# Autodesk Inventor assembly: Assembly1
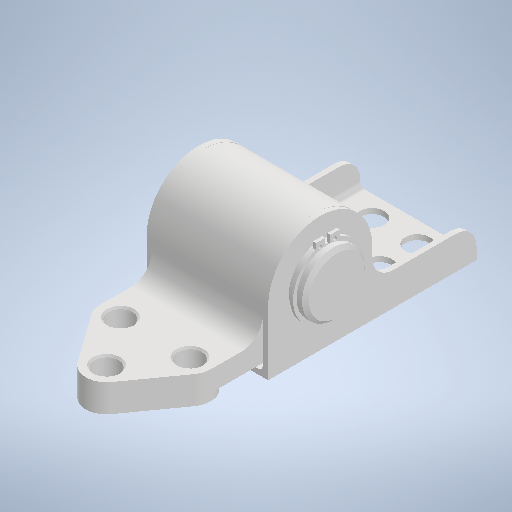
[picture p0: Inventor's stored thumbnail of the model, 512x512]
Saved by Autodesk Inventor 2025 (Build 290162000, 162)
## iProperties
Created: 2025-04-27
Part Number: Assembly1
Document SubType Name: Assembly
Designer: jakub
Author: jakub
## Documents named in this file (5)
- C:\Users\jakub\Documents\Inventor\bitchsdd\Assembly1.iam
- C:\Users\jakub\Documents\Inventor\bitchsdd\AnalniKolicek.ipt
- C:\Users\jakub\Documents\Inventor\bitchsdd\cockring.ipt
- C:\Users\jakub\Documents\Inventor\bitchsdd\num1.ipt
- C:\Users\jakub\Documents\Inventor\bitchsdd\whateverthisis.ipt
## Components (4 placed, 4 different names)
1. AnalniKolicek:1 — Rotational:2, Rotational:3
2. cockring:1 — Rotational:3
3. num1:1 — Rotational:1
4. whateverthisis:1 — Rotational:1, Rotational:2
## Relationships (3: RevoluteJoint 3)
- Rotational:1 [RevoluteJoint] (2.9972 mm): num1:1 ↔ whateverthisis:1
- Rotational:2 [RevoluteJoint] (-9.525 mm): AnalniKolicek:1 ↔ whateverthisis:1
- Rotational:3 [RevoluteJoint]: AnalniKolicek:1 ↔ cockring:1
